# Autodesk Inventor assembly: Assembly - Whole
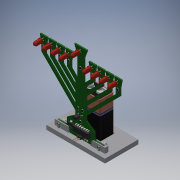
[picture p0: Inventor's stored thumbnail of the model, 180x180]
Saved by Autodesk Inventor 2018.3 (Build 223284000, 284)
## iProperties
Created: 2019-07-24
Part Number: Assembly - Whole
Document SubType Name: Assembly
Designer: Electro707
Author: Electro707
## Documents named in this file (6)
- F:\Projects\UNH MakerSpace Kits\2019 - Winter Holiday\Menourah\CAD-Inventor\Assembly - Whole.iam
- F:\Projects\UNH MakerSpace Kits\2019 - Winter Holiday\Menourah\CAD-Inventor\Holder.ipt
- F:\Projects\UNH MakerSpace Kits\2019 - Winter Holiday\Menourah\CAD-Inventor\Assembly-PCB alone.iam
- C:\Users\Electro707\Documents\Inventor\Content Center Files\R2018\en-US\ANSI B 18.2.4.1 M(1)\ANSI B 18.2.4.1 M - M3 x 0.5Style 1.ipt
- C:\Users\Electro707\Documents\Inventor\Content Center Files\R2018\en-US\IFI 513(3)\IFI 513 - M3x0.5 x 8(2) I.ipt
- F:\Projects\UNH MakerSpace Kits\2019 - Winter Holiday\Menourah\CAD-Inventor\9V Battery.ipt
## Components (7 placed, 5 different names)
1. Holder:1 — Insert:1, Insert:2, Mate:3, Mate:4, Insert:3, Insert:4, Mate:5, Mate:6, Mate:17, Mate:18, Angle:1, Mate:21, Angle:3
2. Assembly-PCB alone:1 [sub-assembly] — Insert:1, Insert:2
3. Hex Nut Metric M3 x 0.5:1 — Mate:4, Mate:6, Mate:9, Mate:10, Mate:14, Mate:15
4. Hex Nut Metric M3 x 0.5:2 — Mate:3, Mate:5, Mate:7, Mate:8, Mate:12, Mate:13
5. Cross Recessed Oval Countersunk Head Machine Screw - Type I - Metric M3x0.5 x 8:1 — Insert:3
6. Cross Recessed Oval Countersunk Head Machine Screw - Type I - Metric M3x0.5 x 8:2 — Insert:4
7. 9V Battery:1 — Mate:17, Mate:19, Angle:2, Mate:22, Angle:4
## Relationships (29: Mate 21, Insert 4, Angle 4)
- Insert:1: Holder:1 ↔ Assembly-PCB alone:1
- Insert:2: Holder:1 ↔ Assembly-PCB alone:1
- Mate:3: Holder:1 ↔ Hex Nut Metric M3 x 0.5:2
- Mate:4: Holder:1 ↔ Hex Nut Metric M3 x 0.5:1
- Insert:3: Holder:1 ↔ Cross Recessed Oval Countersunk Head Machine Screw - Type I - Metric M3x0.5 x 8:1
- Insert:4: Holder:1 ↔ Cross Recessed Oval Countersunk Head Machine Screw - Type I - Metric M3x0.5 x 8:2
- Mate:5: Holder:1 ↔ Hex Nut Metric M3 x 0.5:2
- Mate:6: Holder:1 ↔ Hex Nut Metric M3 x 0.5:1
- Mate:7: Hex Nut Metric M3 x 0.5:2
- Mate:8: Hex Nut Metric M3 x 0.5:2
- Mate:9: Hex Nut Metric M3 x 0.5:1
- Mate:10: Hex Nut Metric M3 x 0.5:1
- Mate:11
- Mate:12: Hex Nut Metric M3 x 0.5:2
- Mate:13: Hex Nut Metric M3 x 0.5:2
- Mate:14: Hex Nut Metric M3 x 0.5:1
- Mate:15: Hex Nut Metric M3 x 0.5:1
- Mate:16
- Mate:17: Holder:1 ↔ 9V Battery:1
- Mate:18: Holder:1
- Angle:1 (0 deg): Holder:1
- Mate:19: 9V Battery:1
- Angle:2 (0 deg): 9V Battery:1
- Mate:20
- Mate:21: Holder:1
- Angle:3 (0 deg): Holder:1
- Mate:22: 9V Battery:1
- Angle:4 (0 deg): 9V Battery:1
- Mate:23
